# Autodesk Inventor assembly: XEnd
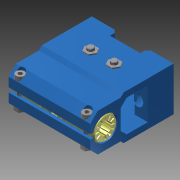
[picture p0: Inventor's stored thumbnail of the model, 180x180]
Saved by Autodesk Inventor 2015 (Build 190159000, 159)
## iProperties
Created: 2014-08-16
Part Number: XEnd
Document SubType Name: Assembly
Designer: Jack
Author: Jack
## Documents named in this file (10)
- C:\Users\Jack\ownCloud\Projects\CoreXY\InventorModel\XAxis\XEnd.iam
- C:\Users\Jack\ownCloud\Projects\CoreXY\InventorModel\XAxis\XEnd.ipt
- C:\Users\Jack\ownCloud\Projects\CoreXY\InventorModel\Hardware\Bearing\Igus\BushingIgusRJM-01-08.ipt
- C:\Users\Jack\ownCloud\Projects\CoreXY\InventorModel\Hardware\Nuts\Nut3.ipt
- C:\Users\Jack\ownCloud\Projects\CoreXY\InventorModel\Hardware\Bolts\SHCS\SHCS3\SHCS3x18.ipt
- C:\Users\Jack\ownCloud\Projects\CoreXY\InventorModel\Hardware\Bolts\SHCS\SHCS4\SHCS4x30.ipt
- C:\Users\Jack\ownCloud\Projects\CoreXY\InventorModel\Hardware\Nuts\Nut4.ipt
- C:\Users\Jack\ownCloud\Projects\CoreXY\InventorModel\Hardware\Bearing\BearingRadialBall\BearingRadialBallF624zz.ipt
- C:\Users\Jack\ownCloud\Projects\CoreXY\InventorModel\Hardware\Wahsers\M4Washer.ipt
- C:\Users\Jack\ownCloud\Projects\CoreXY\InventorModel\Hardware\Bolts\SHCS\SHCS3\SHCS3x8.ipt
## Components (23 placed, 9 different names)
1. XEnd:1 — Mate:1, Mate:2, Mate:3, Mate:4, Mate:5, Mate:6, Mate:7, Mate:8, Mate:9, Angle:1, Angle:2, Mate:10, Mate:11, Mate:13, Mate:15, Mate:16, Mate:17, Mate:18, Mate:19, Angle:3, Angle:4, Mate:22, Mate:23, Mate:31, Mate:39, Mate:40, Mate:41, Angle:5, Angle:6, Mate:44, Mate:45
2. BearingRadialBallF624zz:1
3. BearingRadialBallF624zz:2
4. BearingRadialBallF624zz:3
5. BearingRadialBallF624zz:4
6. M4Washer:4 — Mate:38
7. M4Washer:3 — Mate:39
8. M4Washer:2 — Mate:30, Mate:31
9. M4Washer:1
10. Nut4:2 — Mate:21, Angle:4, Mate:23
11. Nut4:1 — Mate:20, Angle:3, Mate:22
12. SHCS4x30:2 — Mate:17, Mate:18, Mate:20, Mate:38
13. SHCS4x30:1 — Mate:16, Mate:19, Mate:21, Mate:30
14. Nut3:3 — Mate:43, Angle:6, Mate:45, Flush:1
15. Nut3:4 — Mate:42, Angle:5, Mate:44, Flush:2
16. SHCS3x8:1 — Mate:40, Mate:42, Flush:2
17. SHCS3x8:2 — Mate:41, Mate:43, Flush:1
18. SHCS3x18:2 — Mate:14, Mate:15
19. SHCS3x18:1 — Mate:12, Mate:13
20. Nut3:2 — Mate:8, Angle:1, Mate:11, Mate:12
21. Nut3:1 — Mate:9, Angle:2, Mate:10, Mate:14
22. BushingIgusRJM-01-08:2 — Mate:1, Mate:2
23. BushingIgusRJM-01-08:1 — Mate:3, Mate:4
## Relationships (53: Mate 45, Angle 6, Flush 2)
- Mate:1: XEnd:1 ↔ BushingIgusRJM-01-08:2
- Mate:2: XEnd:1 ↔ BushingIgusRJM-01-08:2
- Mate:3: XEnd:1 ↔ BushingIgusRJM-01-08:1
- Mate:4: XEnd:1 ↔ BushingIgusRJM-01-08:1
- Mate:5: XEnd:1
- Mate:6: XEnd:1
- Mate:7: XEnd:1
- Mate:8: XEnd:1 ↔ Nut3:2
- Mate:9: XEnd:1 ↔ Nut3:1
- Angle:1 (0 deg): XEnd:1 ↔ Nut3:2
- Angle:2 (0 deg): XEnd:1 ↔ Nut3:1
- Mate:10: XEnd:1 ↔ Nut3:1
- Mate:11: XEnd:1 ↔ Nut3:2
- Mate:12: SHCS3x18:1 ↔ Nut3:2
- Mate:13: XEnd:1 ↔ SHCS3x18:1
- Mate:14: SHCS3x18:2 ↔ Nut3:1
- Mate:15: XEnd:1 ↔ SHCS3x18:2
- Mate:16: XEnd:1 ↔ SHCS4x30:1
- Mate:17: XEnd:1 ↔ SHCS4x30:2
- Mate:18: XEnd:1 ↔ SHCS4x30:2
- Mate:19: XEnd:1 ↔ SHCS4x30:1
- Mate:20: Nut4:1 ↔ SHCS4x30:2
- Mate:21: Nut4:2 ↔ SHCS4x30:1
- Angle:3 (0 deg): XEnd:1 ↔ Nut4:1
- Angle:4 (0 deg): XEnd:1 ↔ Nut4:2
- Mate:22: XEnd:1 ↔ Nut4:1
- Mate:23: XEnd:1 ↔ Nut4:2
- [Mate]: BearingRadialBallF624zz:1 ↔ BearingRadialBallF624zz:2
- [Mate]: BearingRadialBallF624zz:1 ↔ BearingRadialBallF624zz:2
- [Mate]: BearingRadialBallF624zz:1 ↔ M4Washer:1
- [Mate]: BearingRadialBallF624zz:1 ↔ M4Washer:1
- [Mate]: BearingRadialBallF624zz:2 ↔ M4Washer:2
- [Mate]: BearingRadialBallF624zz:2 ↔ M4Washer:2
- Mate:30: M4Washer:2 ↔ SHCS4x30:1
- Mate:31: XEnd:1 ↔ M4Washer:2
- [Mate]: BearingRadialBallF624zz:3 ↔ BearingRadialBallF624zz:4
- [Mate]: BearingRadialBallF624zz:3 ↔ BearingRadialBallF624zz:4
- [Mate]: BearingRadialBallF624zz:3 ↔ M4Washer:3
- [Mate]: BearingRadialBallF624zz:3 ↔ M4Washer:3
- [Mate]: BearingRadialBallF624zz:4 ↔ M4Washer:4
- [Mate]: BearingRadialBallF624zz:4 ↔ M4Washer:4
- Mate:38: M4Washer:4 ↔ SHCS4x30:2
- Mate:39: XEnd:1 ↔ M4Washer:3
- Mate:40: XEnd:1 ↔ SHCS3x8:1
- Mate:41: XEnd:1 ↔ SHCS3x8:2
- Mate:42: Nut3:4 ↔ SHCS3x8:1
- Mate:43: Nut3:3 ↔ SHCS3x8:2
- Angle:5 (0 deg): XEnd:1 ↔ Nut3:4
- Angle:6 (0 deg): XEnd:1 ↔ Nut3:3
- Mate:44: XEnd:1 ↔ Nut3:4
- Mate:45: XEnd:1 ↔ Nut3:3
- Flush:1 (-0.5 mm): Nut3:3 ↔ SHCS3x8:2
- Flush:2 (-0.5 mm): Nut3:4 ↔ SHCS3x8:1
## Named parameters: d35_d44 = 0 mm, d36_d45 = 0 mm, d37_d46 = 0 mm, d38_d47 = 0 mm, d39_d48 = 0 mm, d40_d49 = 0 mm
